# Autodesk Inventor assembly: xy-mount-asm
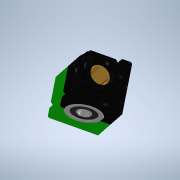
[picture p0: Inventor's stored thumbnail of the model, 180x180]
Saved by Autodesk Inventor 2020.4 (Build 244396000, 396)
## iProperties
Created: 2021-03-01
Part Number: xy-mount-asm
Document SubType Name: Assembly
Designer: AOB
Mass: 44.5102 g
Surface Area: 87.5352 cm^2
Volume: 10.3625 cm^3
Density: 4.29533 g/cm^3
Author: AOB
## Documents named in this file (5)
- C:\Users\marti\Documents\Inventor\ProjectBoron\Boron Ultima\xy-mount-assembly.iam
- C:\Users\marti\Documents\Inventor\ProjectBoron\Boron Ultima\xy-mount-bottom.ipt
- C:\Users\marti\Documents\Inventor\ProjectBoron\Boron Ultima\lm8uu-graphite.ipt
- C:\Users\marti\Documents\Inventor\ProjectBoron\Boron Ultima\688zz bearing.ipt
- C:\Users\marti\Documents\Inventor\ProjectBoron\Boron Ultima\xy-mount-top.ipt
## Components (5 placed, 4 different names)
1. xy-mount-bottom:1 — Cylindrical:1, Cylindrical:2, Mate:1, Flush:3, Mate:2, Mate:3
2. 688zz bearing:1 — Flush:2, Cylindrical:2
3. 688zz bearing:2 — Flush:1, Cylindrical:1
4. xy-mount-top:1 — Mate:1, Flush:3, Mate:4, Flush:2, Flush:1
5. lm8uu-graphite:1 — Mate:2, Mate:3, Mate:4
## Relationships (9: Mate 4, Flush 3, CylindricalJoint 2)
- Flush:1: 688zz bearing:2 ↔ xy-mount-top:1
- Cylindrical:1: xy-mount-bottom:1 ↔ 688zz bearing:2
- Flush:2: 688zz bearing:1 ↔ xy-mount-top:1
- Cylindrical:2: xy-mount-bottom:1 ↔ 688zz bearing:1
- Mate:1: xy-mount-bottom:1 ↔ xy-mount-top:1
- Flush:3: xy-mount-bottom:1 ↔ xy-mount-top:1
- Mate:2: xy-mount-bottom:1 ↔ lm8uu-graphite:1
- Mate:3: xy-mount-bottom:1 ↔ lm8uu-graphite:1
- Mate:4: xy-mount-top:1 ↔ lm8uu-graphite:1
